# Autodesk Inventor assembly: mouse
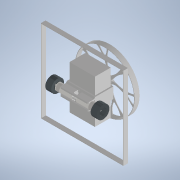
[picture p0: Inventor's stored thumbnail of the model, 180x180]
Saved by Autodesk Inventor 2020 (Build 240168000, 168)
## iProperties
Created: 2020-03-14
Part Number: mouse
Document SubType Name: Assembly
Designer: atmat
Author: atmat
## Documents named in this file (7)
- D:\1.Projects\1.Roboty\5. Micromouse\Czesci\mouse.iam
- D:\1.Projects\1.Roboty\2.JadeJager\Czesci\Ver 1\Motor.ipt
- D:\1.Projects\1.Roboty\5. Micromouse\Czesci\Main.ipt
- D:\1.Projects\1.Roboty\5. Micromouse\Czesci\czujka.ipt
- D:\1.Projects\1.Roboty\5. Micromouse\Czesci\frame.ipt
- D:\1.Projects\1.Roboty\2.JadeJager\Czesci\Ver 1\Wheel.ipt
- D:\1.Projects\1.Roboty\5. Micromouse\Czesci\Koszyk_v2.ipt
## Components (8 placed, 6 different names)
1. Motor:1 — Mate:15, Mate:16, Mate:23, Mate:25, Mate:26
2. Motor:2 — Mate:17, Mate:18, Tangent:1, Mate:22, Mate:23, Mate:27
3. Main:1 — Mate:10, Mate:19, Mate:20, Flush:2, Mate:24
4. czujka:1 — Mate:28, Mate:29
5. frame:1 — Mate:11, Mate:12, Flush:1
6. Wheel:1 — Mate:15, Mate:16
7. Wheel:2 — Mate:17, Mate:18
8. Koszyk_v2:1 — Mate:19, Mate:20, Mate:21, Tangent:1, Mate:22, Mate:25, Mate:26, Mate:27, Mate:28, Mate:29
## Relationships (21: Mate 18, Flush 2, Tangent 1)
- Mate:10 (-48 mm): Main:1
- Mate:11: frame:1
- Mate:12 (90 mm): frame:1
- Flush:1 (90 mm): frame:1
- Mate:15: Motor:1 ↔ Wheel:1
- Mate:16: Motor:1 ↔ Wheel:1
- Mate:17: Motor:2 ↔ Wheel:2
- Mate:18: Motor:2 ↔ Wheel:2
- Mate:19: Main:1 ↔ Koszyk_v2:1
- Mate:20: Main:1 ↔ Koszyk_v2:1
- Mate:21 (-12 mm): Koszyk_v2:1
- Tangent:1: Motor:2 ↔ Koszyk_v2:1
- Mate:22: Motor:2 ↔ Koszyk_v2:1
- Mate:23: Motor:1 ↔ Motor:2
- Flush:2 (-28 mm): Main:1
- Mate:24: Main:1
- Mate:25: Motor:1 ↔ Koszyk_v2:1
- Mate:26: Motor:1 ↔ Koszyk_v2:1
- Mate:27: Motor:2 ↔ Koszyk_v2:1
- Mate:28: czujka:1 ↔ Koszyk_v2:1
- Mate:29 (9 mm): czujka:1 ↔ Koszyk_v2:1
